# Autodesk Inventor assembly: Head
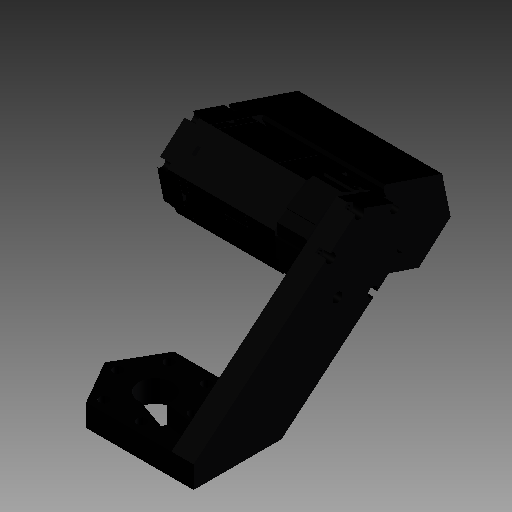
[picture p0: Inventor's stored thumbnail of the model, 512x512]
Saved by Autodesk Inventor 2017 (Build 210142000, 142)
## iProperties
Created: 2018-10-18
Part Number: Head
Document SubType Name: Assembly
Designer: Dell
Author: Dell
## Documents named in this file (5)
- C:\Users\Dell\Documents\GitHub\tr2\Head\Head.iam
- C:\Users\Dell\Documents\GitHub\tr2\Head\Orbbec Astra\Orbbec Astra.iam
- C:\Users\Dell\Documents\GitHub\tr2\Arm Actuator\Arm Actuator.iam
- C:\Users\Dell\Documents\GitHub\tr2\Head\HA07.ipt
- C:\Users\Dell\Documents\GitHub\tr2\Head\HA08.ipt
## Components (4 placed, 4 different names)
1. Orbbec Astra:1 [sub-assembly] — Mate:58, Mate:59, Angle:1
2. Arm Actuator:1 [sub-assembly] — Mate:48, Mate:49, Mate:55, Mate:56, Mate:57
3. HA07:1 — Mate:47, Mate:48, Mate:49, Mate:50, Mate:54
4. HA08:1 — Mate:55, Mate:56, Mate:57, Mate:58, Mate:59, Angle:1
## Relationships (11: Mate 10, Angle 1)
- Mate:47: HA07:1
- Mate:48: Arm Actuator:1 ↔ HA07:1
- Mate:49: Arm Actuator:1 ↔ HA07:1
- Mate:50: HA07:1
- Mate:54: HA07:1
- Mate:55: Arm Actuator:1 ↔ HA08:1
- Mate:56: Arm Actuator:1 ↔ HA08:1
- Mate:57: Arm Actuator:1 ↔ HA08:1
- Mate:58: Orbbec Astra:1 ↔ HA08:1
- Mate:59: Orbbec Astra:1 ↔ HA08:1
- Angle:1 (180 deg): Orbbec Astra:1 ↔ HA08:1
